# Autodesk Inventor assembly: quarter check
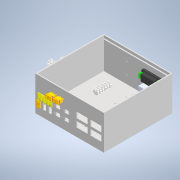
[picture p0: Inventor's stored thumbnail of the model, 180x180]
Saved by Autodesk Inventor 2020.2 (Build 242310000, 310)
## iProperties
Created: 2020-01-17
Part Number: quarter check
Document SubType Name: Assembly
Designer: ColinP
Author: ColinP
## Documents named in this file (10)
- C:\Users\ColinP\Documents\Inventor\HeaterControlIQC\quarter check.iam
- C:\Users\ColinP\Documents\Inventor\HeaterControlIQC\Quarter 2.ipt
- C:\Users\ColinP\Documents\Inventor\HeaterControlIQC\Quarter 3.ipt
- C:\Users\ColinP\Documents\Inventor\HeaterControlIQC\QUarter1.ipt
- C:\Users\ColinP\Documents\Inventor\HeaterControlIQC\Quarter4.ipt
- C:\Users\ColinP\Documents\Inventor\HeaterControlIQC\User Library-Thermocouple_Submini Jack.ipt
- C:\Users\ColinP\Documents\Inventor\HeaterControlIQC\4300-0705.ipt
- C:\Users\ColinP\Documents\Inventor\HeaterControlIQC\06AE2.ipt
- C:\Users\ColinP\Documents\Inventor\HeaterControlIQC\CUI_VSK-S5-5UA-T (1)\CUI_VSK-S5-5UA-T.iam
- C:\Users\ColinP\Documents\Inventor\HeaterControlIQC\OnShore_ES100006DS.ipt
## Components (16 placed, 9 different names)
1. Quarter 2:1 — Mate:5, Mate:6, Flush:1, Flush:4, Mate:27, Mate:28, Mate:29
2. Quarter 3:1 — Mate:3, Mate:4, Mate:5, Flush:2, Flush:4, Mate:7, Mate:8, Mate:9, Mate:10, Mate:11, Mate:12
3. QUarter1:1 — Mate:1, Mate:2, Mate:3, Mate:4, Flush:2, Flush:3
4. Quarter4:1 — Mate:1, Mate:2, Mate:6, Flush:1, Flush:3, Mate:14, Mate:16, Mate:17, Mate:18, Mate:19, Mate:20, Mate:21, Mate:22, Mate:23, Mate:24, Mate:25, Mate:26, Flush:6, Flush:7, Flush:8
5. User Library-Thermocouple_Submini Jack:1 — Mate:16, Mate:17, Mate:18
6. User Library-Thermocouple_Submini Jack:2 — Mate:14, Mate:19, Mate:20
7. User Library-Thermocouple_Submini Jack:3 — Mate:21, Mate:22, Mate:23
8. User Library-Thermocouple_Submini Jack:4 — Mate:24, Mate:25, Mate:26
9. 4300-0705:1
10. 4300-0705:2
11. 4300-0705:3 — Flush:6, Flush:7, Flush:8
12. 06AE2:1 — Mate:10, Mate:11, Mate:12
13. CUI_VSK-S5-5UA-T:1 [sub-assembly] — Mate:7, Mate:8, Mate:9
14. OnShore_ES100006DS:1
15. OnShore_ES100006DS:2
16. OnShore_ES100006DS:3 — Mate:27, Mate:28, Mate:29
## Relationships (34: Mate 27, Flush 7)
- Mate:1: QUarter1:1 ↔ Quarter4:1
- Mate:2: QUarter1:1 ↔ Quarter4:1
- Mate:3: Quarter 3:1 ↔ QUarter1:1
- Mate:4: Quarter 3:1 ↔ QUarter1:1
- Mate:5: Quarter 2:1 ↔ Quarter 3:1
- Mate:6: Quarter 2:1 ↔ Quarter4:1
- Flush:1: Quarter 2:1 ↔ Quarter4:1
- Flush:2: Quarter 3:1 ↔ QUarter1:1
- Flush:3: QUarter1:1 ↔ Quarter4:1
- Flush:4: Quarter 2:1 ↔ Quarter 3:1
- Mate:7: Quarter 3:1 ↔ CUI_VSK-S5-5UA-T:1
- Mate:8: Quarter 3:1 ↔ CUI_VSK-S5-5UA-T:1
- Mate:9: Quarter 3:1 ↔ CUI_VSK-S5-5UA-T:1
- Mate:10: Quarter 3:1 ↔ 06AE2:1
- Mate:11: Quarter 3:1 ↔ 06AE2:1
- Mate:12: Quarter 3:1 ↔ 06AE2:1
- Mate:14: Quarter4:1 ↔ User Library-Thermocouple_Submini Jack:2
- Mate:16: Quarter4:1 ↔ User Library-Thermocouple_Submini Jack:1
- Mate:17: Quarter4:1 ↔ User Library-Thermocouple_Submini Jack:1
- Mate:18: Quarter4:1 ↔ User Library-Thermocouple_Submini Jack:1
- Mate:19: Quarter4:1 ↔ User Library-Thermocouple_Submini Jack:2
- Mate:20: Quarter4:1 ↔ User Library-Thermocouple_Submini Jack:2
- Mate:21: Quarter4:1 ↔ User Library-Thermocouple_Submini Jack:3
- Mate:22: Quarter4:1 ↔ User Library-Thermocouple_Submini Jack:3
- Mate:23: Quarter4:1 ↔ User Library-Thermocouple_Submini Jack:3
- Mate:24: Quarter4:1 ↔ User Library-Thermocouple_Submini Jack:4
- Mate:25: Quarter4:1 ↔ User Library-Thermocouple_Submini Jack:4
- Mate:26: Quarter4:1 ↔ User Library-Thermocouple_Submini Jack:4
- Flush:6: Quarter4:1 ↔ 4300-0705:3
- Flush:7: Quarter4:1 ↔ 4300-0705:3
- Flush:8: Quarter4:1 ↔ 4300-0705:3
- Mate:27: Quarter 2:1 ↔ OnShore_ES100006DS:3
- Mate:28: Quarter 2:1 ↔ OnShore_ES100006DS:3
- Mate:29: Quarter 2:1 ↔ OnShore_ES100006DS:3
